# Autodesk Inventor assembly: Pi
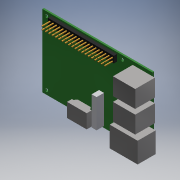
[picture p0: Inventor's stored thumbnail of the model, 180x180]
Saved by Autodesk Inventor 2018 (Build 220112000, 112)
## iProperties
Created: 2018-01-13
Part Number: Pi
Document SubType Name: Assembly
Designer: Kyle-HP
Author: Kyle-HP
## Documents named in this file (8)
- C:\Users\Kyle-HP\Documents\Hackathon-2018\Inventor\Robot\Pi.iam
- C:\Users\Kyle-HP\Documents\Hackathon-2018\Inventor\Robot\PiBoard.ipt
- C:\Users\Kyle-HP\Documents\Hackathon-2018\Inventor\Robot\PiEthernet.ipt
- C:\Users\Kyle-HP\Documents\Hackathon-2018\Inventor\Robot\PiUSB.ipt
- C:\Users\Kyle-HP\Documents\Hackathon-2018\Inventor\Robot\PiHDMI.ipt
- C:\Users\Kyle-HP\Documents\Hackathon-2018\Inventor\Robot\PiGPIOBase.ipt
- C:\Users\Kyle-HP\Documents\Hackathon-2018\Inventor\Robot\PiGPIOPin.ipt
- C:\Users\Kyle-HP\Documents\Hackathon-2018\Inventor\Robot\PiCamera.ipt
## Components (47 placed, 7 different names)
1. PiBoard:1 — Mate:1, Flush:1, Flush:2, Mate:2, Flush:3, Flush:4, Mate:3, Flush:5, Flush:6, Mate:4, Flush:7, Flush:8, Mate:5, Flush:9, Flush:10, Mate:16, Flush:31
2. PiEthernet:1 — Mate:1, Flush:1, Flush:2
3. PiUSB:1 — Mate:3, Flush:5, Flush:6
4. PiUSB:2 — Mate:2, Flush:3, Flush:4
5. PiHDMI:1 — Mate:4, Flush:7, Flush:8, Mate:17
6. PiGPIOBase:1 — Mate:5, Flush:9, Flush:10, Mate:6, Flush:11, Flush:12, Mate:7, Flush:13, Flush:14, Mate:8, Flush:15, Flush:16, Mate:9, Flush:17, Flush:18, Mate:10, Flush:19, Flush:20, Mate:11, Flush:21, Flush:22, Mate:12, Flush:23, Flush:24, Mate:13, Flush:25, Flush:26, Mate:14, Flush:27, Flush:28, Mate:15, Flush:29, Flush:30
7. PiCamera:1 — Mate:16, Flush:31, Mate:17
8. PiGPIOPin:1 — Mate:6, Flush:11, Flush:12
9. PiGPIOPin:2 — Mate:7, Flush:13, Flush:14
10. PiGPIOPin:3 — Mate:8, Flush:15, Flush:16
11. PiGPIOPin:4 — Mate:9, Flush:17, Flush:18
12. PiGPIOPin:5 — Mate:10, Flush:19, Flush:20
13. PiGPIOPin:6 — Mate:11, Flush:21, Flush:22
14. PiGPIOPin:7 — Mate:12, Flush:23, Flush:24
15. PiGPIOPin:8 — Mate:13, Flush:25, Flush:26
16. PiGPIOPin:9 — Mate:14, Flush:27, Flush:28
17. PiGPIOPin:10 — Mate:15, Flush:29, Flush:30
18. PiGPIOPin:11
19. PiGPIOPin:12
20. PiGPIOPin:13
21. PiGPIOPin:14
22. PiGPIOPin:15
23. PiGPIOPin:16
24. PiGPIOPin:17
25. PiGPIOPin:18
26. PiGPIOPin:19
27. PiGPIOPin:20
28. PiGPIOPin:21
29. PiGPIOPin:22
30. PiGPIOPin:23
31. PiGPIOPin:24
32. PiGPIOPin:25
33. PiGPIOPin:26
34. PiGPIOPin:27
35. PiGPIOPin:28
36. PiGPIOPin:29
37. PiGPIOPin:30
38. PiGPIOPin:31
39. PiGPIOPin:32
40. PiGPIOPin:33
41. PiGPIOPin:34
42. PiGPIOPin:35
43. PiGPIOPin:36
44. PiGPIOPin:37
45. PiGPIOPin:38
46. PiGPIOPin:39
47. PiGPIOPin:40
## Component patterns: (4 elements, first: PiGPIOPin:1 + PiGPIOPin:2 + PiGPIOPin:3 + PiGPIOPin:4 + PiGPIOPin:5 + PiGPIOPin:6 + PiGPIOPin:7 + PiGPIOPin:8 + PiGPIOPin:9 + PiGPIOPin:10)
## Relationships (48: Flush 31, Mate 17)
- Mate:1: PiBoard:1 ↔ PiEthernet:1
- Flush:1 (-2.54 mm): PiBoard:1 ↔ PiEthernet:1
- Flush:2 (-2.54 mm): PiBoard:1 ↔ PiEthernet:1
- Mate:2: PiBoard:1 ↔ PiUSB:2
- Flush:3 (22.86 mm): PiBoard:1 ↔ PiUSB:2
- Flush:4 (-1.905 mm): PiBoard:1 ↔ PiUSB:2
- Mate:3: PiBoard:1 ↔ PiUSB:1
- Flush:5 (1.905 mm): PiBoard:1 ↔ PiUSB:1
- Flush:6 (2.54 mm): PiBoard:1 ↔ PiUSB:1
- Mate:4: PiBoard:1 ↔ PiHDMI:1
- Flush:7 (1.905 mm): PiBoard:1 ↔ PiHDMI:1
- Flush:8 (24.765 mm): PiBoard:1 ↔ PiHDMI:1
- Mate:5: PiBoard:1 ↔ PiGPIOBase:1
- Flush:9 (6.985 mm): PiBoard:1 ↔ PiGPIOBase:1
- Flush:10 (1.27 mm): PiBoard:1 ↔ PiGPIOBase:1
- Mate:6: PiGPIOBase:1 ↔ PiGPIOPin:1
- Flush:11 (1.27 mm): PiGPIOBase:1 ↔ PiGPIOPin:1
- Flush:12 (1.27 mm): PiGPIOBase:1 ↔ PiGPIOPin:1
- Mate:7: PiGPIOBase:1 ↔ PiGPIOPin:2
- Flush:13 (1.27 mm): PiGPIOBase:1 ↔ PiGPIOPin:2
- Flush:14 (3.81 mm): PiGPIOBase:1 ↔ PiGPIOPin:2
- Mate:8: PiGPIOBase:1 ↔ PiGPIOPin:3
- Flush:15 (1.27 mm): PiGPIOBase:1 ↔ PiGPIOPin:3
- Flush:16 (6.35 mm): PiGPIOBase:1 ↔ PiGPIOPin:3
- Mate:9: PiGPIOBase:1 ↔ PiGPIOPin:4
- Flush:17 (1.27 mm): PiGPIOBase:1 ↔ PiGPIOPin:4
- Flush:18 (8.89 mm): PiGPIOBase:1 ↔ PiGPIOPin:4
- Mate:10: PiGPIOBase:1 ↔ PiGPIOPin:5
- Flush:19 (1.27 mm): PiGPIOBase:1 ↔ PiGPIOPin:5
- Flush:20 (11.43 mm): PiGPIOBase:1 ↔ PiGPIOPin:5
- Mate:11: PiGPIOBase:1 ↔ PiGPIOPin:6
- Flush:21 (1.27 mm): PiGPIOBase:1 ↔ PiGPIOPin:6
- Flush:22 (13.97 mm): PiGPIOBase:1 ↔ PiGPIOPin:6
- Mate:12: PiGPIOBase:1 ↔ PiGPIOPin:7
- Flush:23 (1.27 mm): PiGPIOBase:1 ↔ PiGPIOPin:7
- Flush:24 (16.51 mm): PiGPIOBase:1 ↔ PiGPIOPin:7
- Mate:13: PiGPIOBase:1 ↔ PiGPIOPin:8
- Flush:25 (1.27 mm): PiGPIOBase:1 ↔ PiGPIOPin:8
- Flush:26 (19.05 mm): PiGPIOBase:1 ↔ PiGPIOPin:8
- Mate:14: PiGPIOBase:1 ↔ PiGPIOPin:9
- Flush:27 (1.27 mm): PiGPIOBase:1 ↔ PiGPIOPin:9
- Flush:28 (21.59 mm): PiGPIOBase:1 ↔ PiGPIOPin:9
- Mate:15: PiGPIOBase:1 ↔ PiGPIOPin:10
- Flush:29 (1.27 mm): PiGPIOBase:1 ↔ PiGPIOPin:10
- Flush:30 (24.13 mm): PiGPIOBase:1 ↔ PiGPIOPin:10
- Mate:16: PiBoard:1 ↔ PiCamera:1
- Flush:31 (1.27 mm): PiBoard:1 ↔ PiCamera:1
- Mate:17 (3.81 mm): PiHDMI:1 ↔ PiCamera:1
